# Autodesk Inventor assembly: Display_Mount_AB
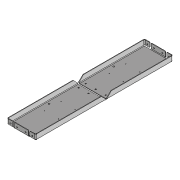
[picture p0: Inventor's stored thumbnail of the model, 180x180]
Saved by Autodesk Inventor 2020 (Build 240168000, 168)
## iProperties
Created: 2021-07-28
Part Number: Display_Mount_AB
Document SubType Name: Assembly
Designer: magnarecta
Author: magnarecta
## Documents named in this file (3)
- C:\Users\lvglv\Documents\GitHub\Eto_Project\Hardware\Parts\Meviy\Meviy_Asem\Display_Mount_AB.iam
- C:\Users\lvglv\Documents\GitHub\Eto_Project\Hardware\Parts\Meviy\Display_Angle.ipt
- C:\Users\lvglv\Documents\GitHub\Eto_Project\Hardware\Parts\Meviy\Display_Angle_B.ipt
## Components (2 placed, 2 different names)
1. Display_Angle:1 — メイト:1, フラッシュ:1, フラッシュ:2
2. Display_Angle_B:1 — メイト:1, フラッシュ:1, フラッシュ:2
## Relationships (3: Flush 2, Mate 1)
- メイト:1 [Mate] (5 mm): Display_Angle:1 ↔ Display_Angle_B:1
- フラッシュ:1 [Flush]: Display_Angle:1 ↔ Display_Angle_B:1
- フラッシュ:2 [Flush]: Display_Angle:1 ↔ Display_Angle_B:1
